# Autodesk Inventor assembly: sole_paint_support
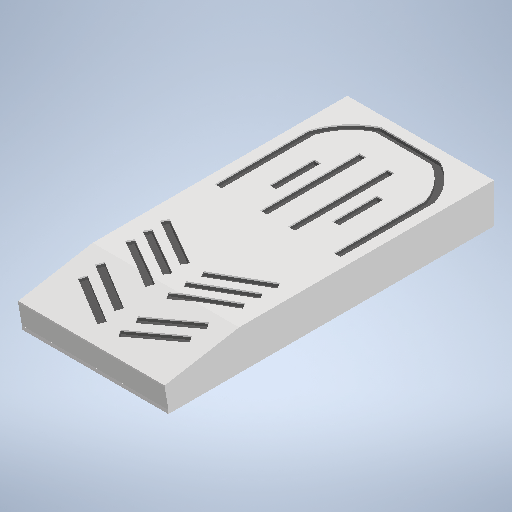
[picture p0: Inventor's stored thumbnail of the model, 512x512]
Saved by Autodesk Inventor 2026.1 (Build 301233020, 233B)
## iProperties
Created: 2026-02-24
Part Number: sole_paint_support
Document SubType Name: Assembly
Designer: hibik
Author: hibik
## Documents named in this file (5)
- C:\Users\hibik\Documents\Robomech\HR\Eglantyne_mark2\hard\leg\sole_paint_support.iam
- C:\Users\hibik\Documents\Robomech\HR\Eglantyne_mark2\hard\leg\toe_sole_bac_big.ipt
- C:\Users\hibik\Documents\Robomech\HR\Eglantyne_mark2\hard\leg\toe_sole_front_big.ipt
- C:\Users\hibik\Documents\Robomech\HR\Eglantyne_mark2\hard\leg\sole_paint_support.ipt
- C:\Users\hibik\Documents\Robomech\HR\Eglantyne_mark2\hard\leg\sole_paint_support_base.ipt
## Components (4 placed, 4 different names)
1. toe_sole_bac_big:1 — フラッシュ:1, フラッシュ:2, メイト:1, 対称度:1, メイト:2, フラッシュ:4
2. toe_sole_front_big:1 — フラッシュ:1, フラッシュ:2, メイト:1, 対称度:1
3. sole_paint_support:1 — フラッシュ:3, メイト:2, フラッシュ:4, フラッシュ:5, フラッシュ:7, フラッシュ:8
4. sole_paint_support_base:1 — フラッシュ:5, フラッシュ:7, フラッシュ:8
## Relationships (10: Flush 7, Mate 2, Symmetry 1)
- フラッシュ:1 [Flush]: toe_sole_bac_big:1 ↔ toe_sole_front_big:1
- フラッシュ:2 [Flush]: toe_sole_bac_big:1 ↔ toe_sole_front_big:1
- メイト:1 [Mate] (3 mm): toe_sole_bac_big:1 ↔ toe_sole_front_big:1
- 対称度:1 [Symmetry]: toe_sole_bac_big:1 ↔ toe_sole_front_big:1
- フラッシュ:3 [Flush]: sole_paint_support:1
- メイト:2 [Mate]: toe_sole_bac_big:1 ↔ sole_paint_support:1
- フラッシュ:4 [Flush]: toe_sole_bac_big:1 ↔ sole_paint_support:1
- フラッシュ:5 [Flush]: sole_paint_support:1 ↔ sole_paint_support_base:1
- フラッシュ:7 [Flush]: sole_paint_support:1 ↔ sole_paint_support_base:1
- フラッシュ:8 [Flush]: sole_paint_support:1 ↔ sole_paint_support_base:1
